# Autodesk Inventor assembly: MTLV-S99
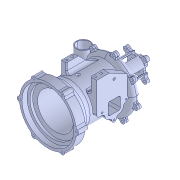
[picture p0: Inventor's stored thumbnail of the model, 180x180]
Saved by Autodesk Inventor 2020 (Build 240168000, 168)
## iProperties
Created: 2020-03-28
Part Number: MTLV-S99
Document SubType Name: Assembly
Designer: John K
Description: TURBINE ASSEMBLY
Author: John K
## Documents named in this file (22)
- C:\GrabCAD\MTL Ventilator Design\MTLV\Subassemblies\MTLV-S99.iam
- C:\GrabCAD\MTL Ventilator Design\MTLV\Manufactured Parts\MTLV-P01.ipt
- C:\GrabCAD\MTL Ventilator Design\MTLV\Manufactured Parts\MTLV-P10.ipt
- C:\GrabCAD\MTL Ventilator Design\MTLV\Manufactured Parts\MTLV-P11.ipt
- C:\GrabCAD\MTL Ventilator Design\MTLV\Manufactured Parts\MTLV-P13.ipt
- C:\GrabCAD\MTL Ventilator Design\MTLV\Commercial Parts\Electronics\Servo Motor HS-322HD.ipt
- C:\GrabCAD\MTL Ventilator Design\MTLV\Manufactured Parts\MTLV-P02.ipt
- C:\GrabCAD\MTL Ventilator Design\MTLV\Commercial Parts\Electronics\Motor\Brushless Motor 2212 920kv.iam
- C:\GrabCAD\MTL Ventilator Design\MTLV\Commercial Parts\Flow-Related\Dust Filter.ipt
- C:\GrabCAD\MTL Ventilator Design\MTLV\Manufactured Parts\MTLV-P12.ipt
- C:\GrabCAD\MTL Ventilator Design\MTLV\Manufactured Parts\MTLV-P09.ipt
- C:\GrabCAD\MTL Ventilator Design\MTLV\Commercial Parts\Electronics\Flow Sensor Digikey SFM3300-250-D.ipt
- C:\GrabCAD\MTL Ventilator Design\MTLV\Commercial Parts\Fasteners\M3x10mm Socket.ipt
- C:\GrabCAD\MTL Ventilator Design\MTLV\Commercial Parts\Fasteners\M4x14mm Socket.ipt
- C:\GrabCAD\MTL Ventilator Design\MTLV\Commercial Parts\Fasteners\M3x6mm Socket.ipt
- C:\GrabCAD\MTL Ventilator Design\MTLV\Commercial Parts\Fasteners\M3 Locknut.ipt
- C:\GrabCAD\MTL Ventilator Design\MTLV\Commercial Parts\Fasteners\M4x16mm Socket.ipt
- C:\GrabCAD\MTL Ventilator Design\MTLV\Manufactured Parts\MTLV-P18.ipt
- C:\GrabCAD\MTL Ventilator Design\MTLV\Commercial Parts\Fasteners\M6 Locknut.ipt
- C:\GrabCAD\MTL Ventilator Design\MTLV\Manufactured Parts\MTLV-P19.ipt
- C:\GrabCAD\MTL Ventilator Design\MTLV\Commercial Parts\Fasteners\M3x25mm Socket.ipt
- C:\GrabCAD\MTL Ventilator Design\MTLV\Manufactured Parts\MTLV-M08.ipt
## Components (57 placed, 21 different names)
1. MTLV-P01:1 — Mate:1, Mate:2, Mate:5, Mate:6, Mate:7, Mate:8, Mate:9, Mate:10, Mate:14, Mate:15, Mate:21, Mate:22, Angle:3, Angle:4, Insert:10, Insert:15, Insert:16, Insert:17, Insert:18, Insert:19, Insert:20, Insert:21, Insert:22, Insert:27, Insert:28, Insert:29, Insert:30, Insert:31, Insert:32, Mate:32, Tangent:1
2. MTLV-P02:1 — Mate:14, Mate:15, Mate:16, Mate:17, Mate:18, Mate:23, Mate:24, Insert:2, Insert:3, Insert:4, Insert:5, Insert:6, Insert:7, Insert:8, Insert:9, Insert:33, Insert:34, Insert:35, Insert:36, Insert:37, Insert:38, Insert:39, Insert:40
3. MTLV-P09:1 — Mate:25, Mate:26, Angle:4, Insert:42, Insert:43
4. MTLV-P10:1 — Mate:1, Mate:2, Mate:3, Angle:1, Mate:4
5. MTLV-P11:1 — Mate:3, Angle:1, Mate:4, Insert:11, Insert:12, Insert:13, Insert:14
6. MTLV-P12:1 — Mate:23, Mate:24, Angle:3, Mate:25, Mate:26, Insert:1
7. MTLV-P13:1 — Mate:5, Mate:6, Mate:7, Mate:11, Mate:12, Mate:13
8. MTLV-P13:2 — Mate:8, Mate:9, Mate:10
9. MTLV-P18:1 — Mate:27, Mate:28, Angle:5, Insert:41, Angle:6
10. MTLV-P19:1 — Mate:29, Mate:30, Mate:31
11. Servo Motor HS-322HD:1 — Mate:11, Mate:12, Mate:13, Insert:23, Insert:24, Insert:25, Insert:26
12. Brushless Motor 2212 920kv:1 [sub-assembly] — Mate:16, Mate:17, Mate:18, Mate:27, Mate:28, Angle:5, Angle:6, Mate:29, Mate:30, Mate:31
13. Dust Filter:1 — Mate:21, Mate:22
14. Flow Sensor Digikey SFM3300-250-D:1 — Insert:1
15. MTLV-M08:1 — Insert:42
16. M3x10mm Socket:19 — Mate:32, Tangent:1
17. M3x6mm Socket:5 — Insert:43
18. M6 Locknut:1 — Insert:41
19. M4x16mm Socket:1 — Insert:23
20. M4x16mm Socket:2 — Insert:24
21. M4x16mm Socket:3 — Insert:25
22. M4x16mm Socket:4 — Insert:26
23. M3x10mm Socket:9 — Insert:27
24. M3x10mm Socket:10 — Insert:28
25. M3x10mm Socket:11 — Insert:29
26. M3x10mm Socket:12 — Insert:30
27. M3x10mm Socket:13 — Insert:31
28. M3x10mm Socket:14 — Insert:32
29. M3x10mm Socket:15 — Insert:33
30. M3x10mm Socket:16 — Insert:34
31. M3x10mm Socket:17 — Insert:35
32. M3x10mm Socket:18 — Insert:36
33. M3x25mm Socket:1 — Insert:37
34. M3x25mm Socket:2 — Insert:38
35. M3x25mm Socket:3 — Insert:40
36. M3x25mm Socket:4 — Insert:39
37. M3x10mm Socket:1 — Insert:2
38. M3x10mm Socket:2 — Insert:3
39. M3x10mm Socket:3 — Insert:4
40. M3x10mm Socket:4 — Insert:5
41. M3x10mm Socket:5 — Insert:6
42. M3x10mm Socket:6 — Insert:7
43. M3x10mm Socket:7 — Insert:8
44. M3x10mm Socket:8 — Insert:9
45. M4x14mm Socket:1 — Insert:10
46. M3x6mm Socket:1 — Insert:11
47. M3x6mm Socket:2 — Insert:12
48. M3x6mm Socket:3 — Insert:13
49. M3x6mm Socket:4 — Insert:14
50. M3 Locknut:1 — Insert:15
51. M3 Locknut:2 — Insert:16
52. M3 Locknut:3 — Insert:17
53. M3 Locknut:4 — Insert:18
54. M3 Locknut:5 — Insert:19
55. M3 Locknut:6 — Insert:20
56. M3 Locknut:7 — Insert:21
57. M3 Locknut:8 — Insert:22
## Relationships (79: Insert 43, Mate 30, Angle 5, Tangent 1)
- Mate:1: MTLV-P01:1 ↔ MTLV-P10:1
- Mate:2: MTLV-P01:1 ↔ MTLV-P10:1
- Mate:3: MTLV-P10:1 ↔ MTLV-P11:1
- Angle:1 (0 deg): MTLV-P10:1 ↔ MTLV-P11:1
- Mate:4: MTLV-P10:1 ↔ MTLV-P11:1
- Mate:5: MTLV-P01:1 ↔ MTLV-P13:1
- Mate:6: MTLV-P01:1 ↔ MTLV-P13:1
- Mate:7: MTLV-P01:1 ↔ MTLV-P13:1
- Mate:8: MTLV-P01:1 ↔ MTLV-P13:2
- Mate:9: MTLV-P01:1 ↔ MTLV-P13:2
- Mate:10: MTLV-P01:1 ↔ MTLV-P13:2
- Mate:11: MTLV-P13:1 ↔ Servo Motor HS-322HD:1
- Mate:12: MTLV-P13:1 ↔ Servo Motor HS-322HD:1
- Mate:13: MTLV-P13:1 ↔ Servo Motor HS-322HD:1
- Mate:14: MTLV-P01:1 ↔ MTLV-P02:1
- Mate:15: MTLV-P01:1 ↔ MTLV-P02:1
- Mate:16: MTLV-P02:1 ↔ Brushless Motor 2212 920kv:1
- Mate:17 (17.3 mm): MTLV-P02:1 ↔ Brushless Motor 2212 920kv:1
- Mate:18: MTLV-P02:1 ↔ Brushless Motor 2212 920kv:1
- Mate:21: MTLV-P01:1 ↔ Dust Filter:1
- Mate:22: MTLV-P01:1 ↔ Dust Filter:1
- Mate:23: MTLV-P02:1 ↔ MTLV-P12:1
- Mate:24: MTLV-P02:1 ↔ MTLV-P12:1
- Angle:3 (0 deg): MTLV-P01:1 ↔ MTLV-P12:1
- Mate:25: MTLV-P09:1 ↔ MTLV-P12:1
- Mate:26: MTLV-P09:1 ↔ MTLV-P12:1
- Angle:4 (0 deg): MTLV-P01:1 ↔ MTLV-P09:1
- Insert:1: MTLV-P12:1 ↔ Flow Sensor Digikey SFM3300-250-D:1
- Insert:2: MTLV-P02:1 ↔ M3x10mm Socket:1
- Insert:3: MTLV-P02:1 ↔ M3x10mm Socket:2
- Insert:4: MTLV-P02:1 ↔ M3x10mm Socket:3
- Insert:5: MTLV-P02:1 ↔ M3x10mm Socket:4
- Insert:6: MTLV-P02:1 ↔ M3x10mm Socket:5
- Insert:7: MTLV-P02:1 ↔ M3x10mm Socket:6
- Insert:8: MTLV-P02:1 ↔ M3x10mm Socket:7
- Insert:9: MTLV-P02:1 ↔ M3x10mm Socket:8
- Insert:10: MTLV-P01:1 ↔ M4x14mm Socket:1
- Insert:11: MTLV-P11:1 ↔ M3x6mm Socket:1
- Insert:12: MTLV-P11:1 ↔ M3x6mm Socket:2
- Insert:13: MTLV-P11:1 ↔ M3x6mm Socket:3
- Insert:14: MTLV-P11:1 ↔ M3x6mm Socket:4
- Insert:15: MTLV-P01:1 ↔ M3 Locknut:1
- Insert:16: MTLV-P01:1 ↔ M3 Locknut:2
- Insert:17: MTLV-P01:1 ↔ M3 Locknut:3
- Insert:18: MTLV-P01:1 ↔ M3 Locknut:4
- Insert:19: MTLV-P01:1 ↔ M3 Locknut:5
- Insert:20: MTLV-P01:1 ↔ M3 Locknut:6
- Insert:21: MTLV-P01:1 ↔ M3 Locknut:7
- Insert:22: MTLV-P01:1 ↔ M3 Locknut:8
- Insert:23: Servo Motor HS-322HD:1 ↔ M4x16mm Socket:1
- Insert:24: Servo Motor HS-322HD:1 ↔ M4x16mm Socket:2
- Insert:25: Servo Motor HS-322HD:1 ↔ M4x16mm Socket:3
- Insert:26: Servo Motor HS-322HD:1 ↔ M4x16mm Socket:4
- Insert:27 (4.1 mm): MTLV-P01:1 ↔ M3x10mm Socket:9
- Insert:28 (4.1 mm): MTLV-P01:1 ↔ M3x10mm Socket:10
- Insert:29 (4.1 mm): MTLV-P01:1 ↔ M3x10mm Socket:11
- Insert:30 (4.1 mm): MTLV-P01:1 ↔ M3x10mm Socket:12
- Insert:31 (4.1 mm): MTLV-P01:1 ↔ M3x10mm Socket:13
- Insert:32 (4.1 mm): MTLV-P01:1 ↔ M3x10mm Socket:14
- Insert:33 (4.1 mm): MTLV-P02:1 ↔ M3x10mm Socket:15
- Insert:34 (4.1 mm): MTLV-P02:1 ↔ M3x10mm Socket:16
- Insert:35 (4.1 mm): MTLV-P02:1 ↔ M3x10mm Socket:17
- Insert:36 (4.1 mm): MTLV-P02:1 ↔ M3x10mm Socket:18
- Insert:37: MTLV-P02:1 ↔ M3x25mm Socket:1
- Insert:38: MTLV-P02:1 ↔ M3x25mm Socket:2
- Insert:39: MTLV-P02:1 ↔ M3x25mm Socket:4
- Insert:40: MTLV-P02:1 ↔ M3x25mm Socket:3
- Mate:27: MTLV-P18:1 ↔ Brushless Motor 2212 920kv:1
- Mate:28: MTLV-P18:1 ↔ Brushless Motor 2212 920kv:1
- Angle:5 (180 deg): MTLV-P18:1 ↔ Brushless Motor 2212 920kv:1
- Insert:41: MTLV-P18:1 ↔ M6 Locknut:1
- Angle:6 (180 deg): MTLV-P18:1 ↔ Brushless Motor 2212 920kv:1
- Mate:29: MTLV-P19:1 ↔ Brushless Motor 2212 920kv:1
- Mate:30: MTLV-P19:1 ↔ Brushless Motor 2212 920kv:1
- Mate:31: MTLV-P19:1 ↔ Brushless Motor 2212 920kv:1
- Insert:42: MTLV-P09:1 ↔ MTLV-M08:1
- Insert:43: MTLV-P09:1 ↔ M3x6mm Socket:5
- Mate:32: MTLV-P01:1 ↔ M3x10mm Socket:19
- Tangent:1: MTLV-P01:1 ↔ M3x10mm Socket:19
